# Autodesk Inventor assembly: 000.011 - Крепление по XT60 мама
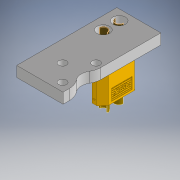
[picture p0: Inventor's stored thumbnail of the model, 180x180]
Saved by Autodesk Inventor 2022 (Build 260153000, 153)
## iProperties
Created: 2023-04-23
Part Number: 000.011 - Крепление по XT60 мама
Document SubType Name: Assembly
Designer: Иван Петров
Author: Иван Петров
## Documents named in this file (4)
- C:\Users\Ivan Petrov\Documents\GitHub\OmniBot\design\000.011 - Крепление по XT60 мама.iam
- C:\Users\Ivan Petrov\Documents\GitHub\OmniBot\design\000.011.001 - Основание.ipt
- C:\Users\Ivan Petrov\Documents\GitHub\OmniBot\design\standart_components\XT60 Buchse.ipt
- C:\Users\Ivan Petrov\Documents\GitHub\OmniBot\design\standart_components\XT60FemaleConnector.ipt
## Components (3 placed, 3 different names)
1. 000.011.001 - Основание:1 — Совмещение:2, Совмещение:3, Совмещение:4
2. XT60 Buchse:1 — Совмещение:1, Совмещение:2, Совмещение:3, Совмещение:4, Совмещение:5, Угол:1
3. XT60FemaleConnector:1 — Совмещение:1, Совмещение:5, Угол:1
## Relationships (6: Mate 5, Angle 1)
- Совмещение:1 [Mate]: XT60 Buchse:1 ↔ XT60FemaleConnector:1
- Совмещение:2 [Mate]: 000.011.001 - Основание:1 ↔ XT60 Buchse:1
- Совмещение:3 [Mate]: 000.011.001 - Основание:1 ↔ XT60 Buchse:1
- Совмещение:4 [Mate]: 000.011.001 - Основание:1 ↔ XT60 Buchse:1
- Совмещение:5 [Mate]: XT60 Buchse:1 ↔ XT60FemaleConnector:1
- Угол:1 [Angle] (0 deg): XT60 Buchse:1 ↔ XT60FemaleConnector:1
